# Autodesk Inventor assembly: Storage Rack Assembly
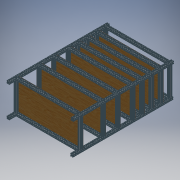
[picture p0: Inventor's stored thumbnail of the model, 180x180]
Saved by Autodesk Inventor 2019.4 (Build 234330000, 330)
## iProperties
Created: 2020-02-27
Part Number: Storage Rack Assembly
Document SubType Name: Assembly
Designer: admin
Author: admin
## Documents named in this file (5)
- C:\Users\admin\Desktop\FRC 2020 Engineering\GitHub\7738-2020\Pit Station Designs\Storage racks\Storage Rack Assembly.iam
- C:\Users\admin\Desktop\FRC 2020 Engineering\GitHub\7738-2020\Pit Station Designs\Storage racks\Storage Rack Legs.ipt
- C:\Users\admin\Desktop\FRC 2020 Engineering\GitHub\7738-2020\Pit Station Designs\Storage racks\Cross beams.ipt
- C:\Users\admin\Desktop\FRC 2020 Engineering\GitHub\7738-2020\Pit Station Designs\Storage racks\Cross beams short.ipt
- C:\Users\admin\Desktop\FRC 2020 Engineering\GitHub\7738-2020\Pit Station Designs\Storage racks\Wooden Rack Plate.ipt
## Components (43 placed, 4 different names)
1. Storage Rack Legs:2 — Mate:3, Mate:16, Flush:9
2. Storage Rack Legs:3 — Mate:2, Mate:5, Mate:6, Mate:7, Mate:8, Mate:9, Flush:1, Flush:2, Flush:3, Flush:4, Flush:5, Flush:6, Mate:14, Flush:7, Flush:8, Mate:15, Mate:19, Flush:10, Flush:29, Flush:30, Mate:53
3. Cross beams:1 — Mate:6, Flush:3, Mate:10, Mate:11
4. Cross beams:2 — Mate:5, Flush:1, Flush:2, Mate:10, Mate:54
5. Cross beams:3 — Mate:7, Flush:4, Mate:11, Mate:12
6. Cross beams:4 — Mate:8, Flush:5, Mate:12, Mate:13
7. Cross beams:5 — Mate:9, Flush:6, Mate:13, Mate:17
8. Cross beams:6 — Mate:14, Flush:7, Mate:17, Mate:18
9. Cross beams:7 — Flush:8, Mate:15, Mate:16, Flush:9, Mate:18, Mate:20
10. Cross beams:8 — Mate:19, Flush:10, Mate:20
11. Storage Rack Legs:4 — Mate:45, Mate:46, Mate:47, Mate:48, Mate:49, Mate:50, Mate:51, Mate:52, Flush:39, Flush:40, Flush:41, Flush:42, Flush:43, Flush:44, Flush:45, Flush:46, Mate:68, Mate:69, Mate:70, Mate:71, Mate:72, Mate:73, Mate:74
12. Storage Rack Legs:5 — Mate:37, Mate:38, Mate:39, Mate:40, Mate:41, Mate:42, Mate:43, Mate:44, Flush:21, Flush:22, Flush:23, Flush:24, Flush:25, Flush:26, Flush:27, Flush:28, Flush:29, Mate:61, Mate:62, Mate:63, Mate:64, Mate:65, Mate:66, Mate:67
13. Cross beams:9 — Flush:37, Flush:53, Mate:55
14. Cross beams:10 — Flush:38, Flush:54
15. Cross beams:11 — Flush:36, Flush:52, Mate:56
16. Cross beams:12 — Flush:35, Flush:51
17. Cross beams:13 — Flush:34, Flush:50, Mate:58
18. Cross beams:14 — Flush:33, Flush:49, Mate:59
19. Cross beams:15 — Flush:32, Flush:48
20. Cross beams:16 — Flush:31, Flush:47
21. Cross beams short:1 — Mate:44, Flush:28, Flush:30, Mate:53, Flush:31
22. Cross beams short:2 — Mate:43, Flush:27, Flush:32
23. Cross beams short:3 — Mate:42, Flush:26, Flush:33
24. Cross beams short:4 — Mate:41, Flush:25, Flush:34
25. Cross beams short:5 — Mate:40, Flush:24, Flush:35
26. Cross beams short:6 — Mate:39, Flush:23, Flush:36
27. Cross beams short:7 — Mate:38, Flush:22, Flush:37
28. Cross beams short:8 — Mate:37, Flush:21, Flush:38
29. Cross beams short:9 — Mate:45, Flush:46, Flush:47
30. Cross beams short:10 — Mate:46, Flush:45, Flush:48, Mate:60
31. Cross beams short:11 — Mate:47, Flush:44, Flush:49
32. Cross beams short:12 — Mate:48, Flush:43, Flush:50
33. Cross beams short:13 — Mate:49, Flush:42, Flush:51, Mate:57
34. Cross beams short:14 — Mate:50, Flush:41, Flush:52
35. Cross beams short:15 — Mate:51, Flush:40, Flush:53
36. Cross beams short:16 — Mate:52, Flush:39, Flush:54
37. Wooden Rack Plate:1 — Mate:54, Mate:62, Mate:74
38. Wooden Rack Plate:2 — Mate:55, Mate:63, Mate:73
39. Wooden Rack Plate:3 — Mate:56, Mate:64, Mate:72
40. Wooden Rack Plate:4 — Mate:57, Mate:65, Mate:71
41. Wooden Rack Plate:5 — Mate:58, Mate:66, Mate:70
42. Wooden Rack Plate:6 — Mate:59, Mate:67, Mate:69
43. Wooden Rack Plate:7 — Mate:60, Mate:61, Mate:68
## Relationships (126: Mate 72, Flush 54)
- Mate:2: Storage Rack Legs:3
- Mate:3: Storage Rack Legs:2
- Mate:5: Storage Rack Legs:3 ↔ Cross beams:2
- Mate:6: Storage Rack Legs:3 ↔ Cross beams:1
- Mate:7: Storage Rack Legs:3 ↔ Cross beams:3
- Mate:8: Storage Rack Legs:3 ↔ Cross beams:4
- Mate:9: Storage Rack Legs:3 ↔ Cross beams:5
- Flush:1 (100 mm): Storage Rack Legs:3 ↔ Cross beams:2
- Flush:2: Storage Rack Legs:3 ↔ Cross beams:2
- Flush:3: Storage Rack Legs:3 ↔ Cross beams:1
- Flush:4: Storage Rack Legs:3 ↔ Cross beams:3
- Flush:5: Storage Rack Legs:3 ↔ Cross beams:4
- Flush:6: Storage Rack Legs:3 ↔ Cross beams:5
- Mate:10 (300 mm): Cross beams:1 ↔ Cross beams:2
- Mate:11 (180 mm): Cross beams:1 ↔ Cross beams:3
- Mate:12 (180 mm): Cross beams:3 ↔ Cross beams:4
- Mate:13 (100 mm): Cross beams:4 ↔ Cross beams:5
- Mate:14: Storage Rack Legs:3 ↔ Cross beams:6
- Flush:7: Storage Rack Legs:3 ↔ Cross beams:6
- Flush:8: Storage Rack Legs:3 ↔ Cross beams:7
- Mate:15: Storage Rack Legs:3 ↔ Cross beams:7
- Mate:16: Storage Rack Legs:2 ↔ Cross beams:7
- Flush:9: Storage Rack Legs:2 ↔ Cross beams:7
- Mate:17 (100 mm): Cross beams:5 ↔ Cross beams:6
- Mate:18 (100 mm): Cross beams:6 ↔ Cross beams:7
- Mate:19: Storage Rack Legs:3 ↔ Cross beams:8
- Flush:10: Storage Rack Legs:3 ↔ Cross beams:8
- Mate:20 (100 mm): Cross beams:7 ↔ Cross beams:8
- [Mate]: Storage Rack Legs:5 ↔ Cross beams:10
- [Mate]: Storage Rack Legs:5 ↔ Cross beams:9
- [Mate]: Storage Rack Legs:5 ↔ Cross beams:11
- [Mate]: Storage Rack Legs:5 ↔ Cross beams:12
- [Mate]: Storage Rack Legs:5 ↔ Cross beams:13
- [Flush] (100 mm): Storage Rack Legs:5 ↔ Cross beams:10
- [Flush]: Storage Rack Legs:5 ↔ Cross beams:10
- [Flush]: Storage Rack Legs:5 ↔ Cross beams:9
- [Flush]: Storage Rack Legs:5 ↔ Cross beams:11
- [Flush]: Storage Rack Legs:5 ↔ Cross beams:12
- [Flush]: Storage Rack Legs:5 ↔ Cross beams:13
- [Mate] (300 mm): Cross beams:9 ↔ Cross beams:10
- [Mate] (180 mm): Cross beams:9 ↔ Cross beams:11
- [Mate] (180 mm): Cross beams:11 ↔ Cross beams:12
- [Mate] (100 mm): Cross beams:12 ↔ Cross beams:13
- [Mate]: Storage Rack Legs:5 ↔ Cross beams:14
- [Flush]: Storage Rack Legs:5 ↔ Cross beams:14
- [Flush]: Storage Rack Legs:5 ↔ Cross beams:15
- [Mate]: Storage Rack Legs:5 ↔ Cross beams:15
- [Mate]: Storage Rack Legs:4 ↔ Cross beams:15
- [Flush]: Storage Rack Legs:4 ↔ Cross beams:15
- [Mate] (100 mm): Cross beams:13 ↔ Cross beams:14
- [Mate] (100 mm): Cross beams:14 ↔ Cross beams:15
- [Mate]: Storage Rack Legs:5 ↔ Cross beams:16
- [Flush]: Storage Rack Legs:5 ↔ Cross beams:16
- [Mate] (100 mm): Cross beams:15 ↔ Cross beams:16
- Mate:37: Storage Rack Legs:5 ↔ Cross beams short:8
- Mate:38: Storage Rack Legs:5 ↔ Cross beams short:7
- Mate:39: Storage Rack Legs:5 ↔ Cross beams short:6
- Mate:40: Storage Rack Legs:5 ↔ Cross beams short:5
- Mate:41: Storage Rack Legs:5 ↔ Cross beams short:4
- Mate:42: Storage Rack Legs:5 ↔ Cross beams short:3
- Mate:43: Storage Rack Legs:5 ↔ Cross beams short:2
- Mate:44: Storage Rack Legs:5 ↔ Cross beams short:1
- Mate:45: Storage Rack Legs:4 ↔ Cross beams short:9
- Mate:46: Storage Rack Legs:4 ↔ Cross beams short:10
- Mate:47: Storage Rack Legs:4 ↔ Cross beams short:11
- Mate:48: Storage Rack Legs:4 ↔ Cross beams short:12
- Mate:49: Storage Rack Legs:4 ↔ Cross beams short:13
- Mate:50: Storage Rack Legs:4 ↔ Cross beams short:14
- Mate:51: Storage Rack Legs:4 ↔ Cross beams short:15
- Mate:52: Storage Rack Legs:4 ↔ Cross beams short:16
- Flush:21: Storage Rack Legs:5 ↔ Cross beams short:8
- Flush:22: Storage Rack Legs:5 ↔ Cross beams short:7
- Flush:23: Storage Rack Legs:5 ↔ Cross beams short:6
- Flush:24: Storage Rack Legs:5 ↔ Cross beams short:5
- Flush:25: Storage Rack Legs:5 ↔ Cross beams short:4
- Flush:26: Storage Rack Legs:5 ↔ Cross beams short:3
- Flush:27: Storage Rack Legs:5 ↔ Cross beams short:2
- Flush:28: Storage Rack Legs:5 ↔ Cross beams short:1
- Flush:29: Storage Rack Legs:3 ↔ Storage Rack Legs:5
- Flush:30: Storage Rack Legs:3 ↔ Cross beams short:1
- Mate:53: Storage Rack Legs:3 ↔ Cross beams short:1
- Flush:31: Cross beams:16 ↔ Cross beams short:1
- Flush:32: Cross beams:15 ↔ Cross beams short:2
- Flush:33: Cross beams:14 ↔ Cross beams short:3
- Flush:34: Cross beams:13 ↔ Cross beams short:4
- Flush:35: Cross beams:12 ↔ Cross beams short:5
- Flush:36: Cross beams:11 ↔ Cross beams short:6
- Flush:37: Cross beams:9 ↔ Cross beams short:7
- Flush:38: Cross beams:10 ↔ Cross beams short:8
- Flush:39: Storage Rack Legs:4 ↔ Cross beams short:16
- Flush:40: Storage Rack Legs:4 ↔ Cross beams short:15
- Flush:41: Storage Rack Legs:4 ↔ Cross beams short:14
- Flush:42: Storage Rack Legs:4 ↔ Cross beams short:13
- Flush:43: Storage Rack Legs:4 ↔ Cross beams short:12
- Flush:44: Storage Rack Legs:4 ↔ Cross beams short:11
- Flush:45: Storage Rack Legs:4 ↔ Cross beams short:10
- Flush:46: Storage Rack Legs:4 ↔ Cross beams short:9
- Flush:47: Cross beams:16 ↔ Cross beams short:9
- Flush:48: Cross beams:15 ↔ Cross beams short:10
- Flush:49: Cross beams:14 ↔ Cross beams short:11
- Flush:50: Cross beams:13 ↔ Cross beams short:12
- Flush:51: Cross beams:12 ↔ Cross beams short:13
- Flush:52: Cross beams:11 ↔ Cross beams short:14
- Flush:53: Cross beams:9 ↔ Cross beams short:15
- Flush:54: Cross beams:10 ↔ Cross beams short:16
- Mate:54: Cross beams:2 ↔ Wooden Rack Plate:1
- Mate:55: Cross beams:9 ↔ Wooden Rack Plate:2
- Mate:56: Cross beams:11 ↔ Wooden Rack Plate:3
- Mate:57: Cross beams short:13 ↔ Wooden Rack Plate:4
- Mate:58: Cross beams:13 ↔ Wooden Rack Plate:5
- Mate:59: Cross beams:14 ↔ Wooden Rack Plate:6
- Mate:60: Cross beams short:10 ↔ Wooden Rack Plate:7
- Mate:61 (2 mm): Storage Rack Legs:5 ↔ Wooden Rack Plate:7
- Mate:62 (2 mm): Storage Rack Legs:5 ↔ Wooden Rack Plate:1
- Mate:63 (2 mm): Storage Rack Legs:5 ↔ Wooden Rack Plate:2
- Mate:64 (2 mm): Storage Rack Legs:5 ↔ Wooden Rack Plate:3
- Mate:65 (2 mm): Storage Rack Legs:5 ↔ Wooden Rack Plate:4
- Mate:66 (2 mm): Storage Rack Legs:5 ↔ Wooden Rack Plate:5
- Mate:67 (2 mm): Storage Rack Legs:5 ↔ Wooden Rack Plate:6
- Mate:68 (2 mm): Storage Rack Legs:4 ↔ Wooden Rack Plate:7
- Mate:69 (2 mm): Storage Rack Legs:4 ↔ Wooden Rack Plate:6
- Mate:70 (2 mm): Storage Rack Legs:4 ↔ Wooden Rack Plate:5
- Mate:71 (2 mm): Storage Rack Legs:4 ↔ Wooden Rack Plate:4
- Mate:72 (2 mm): Storage Rack Legs:4 ↔ Wooden Rack Plate:3
- Mate:73 (2 mm): Storage Rack Legs:4 ↔ Wooden Rack Plate:2
- Mate:74 (2 mm): Storage Rack Legs:4 ↔ Wooden Rack Plate:1
## Named parameters: d35_d33 = 0 mm, d36_d34 = 100 mm, d37_d25 = 0 mm, d38_d26 = 0 mm, d39_d28 = 0 mm, d40_d29 = 0 mm, d41_d30 = 100 mm, d42_d31 = 100 mm, d43_d32 = 0 mm, d44_d21 = 0 mm, d45_d24 = 0 mm, d46_d15 = 300 mm, d47_d16 = 180 mm, d48_d17 = 180 mm, d49_d18 = 100 mm, d50_d4 = 0 mm, d51_d5 = 0 mm, d52_d6 = 0 mm, d53_d7 = 0 mm, d54_d8 = 0 mm, d55_d9 = 100 mm, d56_d10 = 0 mm, d57_d11 = 0 mm, d58_d12 = 0 mm, d59_d13 = 0 mm, d60_d14 = 0 mm
